# Autodesk Inventor assembly: Electromagnetic cover
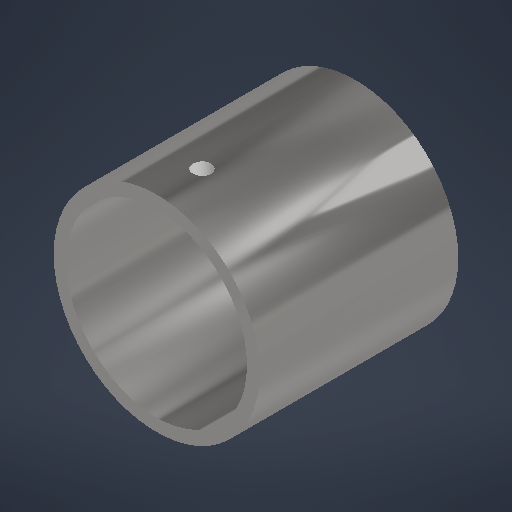
[picture p0: Inventor's stored thumbnail of the model, 512x512]
Saved by Autodesk Inventor 2026.3 (Build 303398000, 398)
## iProperties
Created: 2026-08-03
Part Number: Electromagnetic cover
Document SubType Name: Assembly
Designer: matot
Author: matot
## Documents named in this file (3)
- C:\Users\matot\OneDrive - Stellenbosch University\2026\MechatronicsProject478\Building the joint\Joint Assembly\Electromagnetic cover.iam
- C:\Users\matot\OneDrive - Stellenbosch University\2026\MechatronicsProject478\Building the joint\Joint Assembly\Electromagnetic cover body.ipt
- C:\Users\matot\OneDrive - Stellenbosch University\2026\MechatronicsProject478\Building the joint\Joint Assembly\Electromagnetic cover bottom.ipt
## Components (2 placed, 2 different names)
1. Electromagnetic cover body:2 — Insert:1
2. Electromagnetic cover bottom:1 — Insert:1
## Relationships (1: Insert 1)
- Insert:1: Electromagnetic cover body:2 ↔ Electromagnetic cover bottom:1
